# Autodesk Inventor assembly: Toolhead
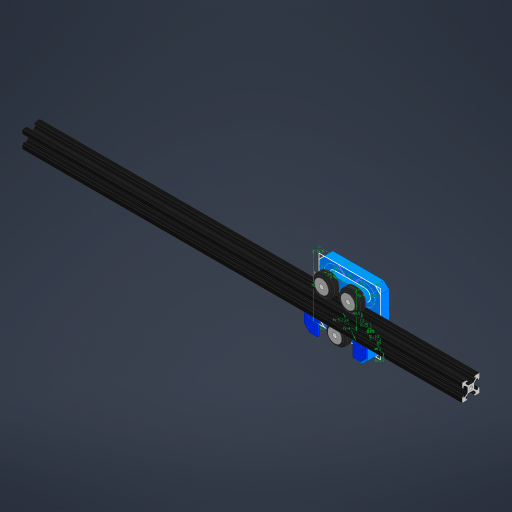
[picture p0: Inventor's stored thumbnail of the model, 512x512]
Saved by Autodesk Inventor 2024.2 (Build 282272000, 272)
## iProperties
Created: 2024-10-17
Part Number: Toolhead
Document SubType Name: Assembly
Designer: jerem
Author: jerem
## Documents named in this file (5)
- C:\Users\jerem\Documents\GitHub\Perovskite-Automated-Synthesis-System\CAD\Gantry\Toolhead\Toolhead.iam
- C:\Users\jerem\Documents\GitHub\Perovskite-Automated-Synthesis-System\CAD\Gantry\Extrusion\V Extrustion 20x500mm.ipt
- C:\Users\jerem\Documents\GitHub\Perovskite-Automated-Synthesis-System\CAD\Gantry\Printer Wheel.ipt
- C:\Users\jerem\Documents\GitHub\Perovskite-Automated-Synthesis-System\CAD\Gantry\Toolhead\Toolhead Base.ipt
- C:\Users\jerem\Documents\GitHub\Perovskite-Automated-Synthesis-System\CAD\Gantry\Toolhead\Belt Holders.ipt
## Components (7 placed, 4 different names)
1. V Extrustion 20x500mm:1 — Mate:7, Flush:1
2. Printer Wheel:1 — Mate:2, Mate:5
3. Printer Wheel:2 — Mate:3, Mate:6, Mate:7
4. Printer Wheel:3 — Mate:1, Mate:4
5. Toolhead Base:1 — Mate:1, Mate:2, Mate:3, Mate:4, Mate:5, Mate:6, Flush:1, Mate:8, Mate:9, Mate:10, Mate:11, Mate:12, Mate:13
6. Belt Holders:1 — Mate:8, Mate:9, Mate:10
7. Belt Holders:2 — Mate:11, Mate:12, Mate:13
## Relationships (14: Mate 13, Flush 1)
- Mate:1: Printer Wheel:3 ↔ Toolhead Base:1
- Mate:2: Printer Wheel:1 ↔ Toolhead Base:1
- Mate:3: Printer Wheel:2 ↔ Toolhead Base:1
- Mate:4: Printer Wheel:3 ↔ Toolhead Base:1
- Mate:5: Printer Wheel:1 ↔ Toolhead Base:1
- Mate:6: Printer Wheel:2 ↔ Toolhead Base:1
- Mate:7: V Extrustion 20x500mm:1 ↔ Printer Wheel:2
- Flush:1: V Extrustion 20x500mm:1 ↔ Toolhead Base:1
- Mate:8: Toolhead Base:1 ↔ Belt Holders:1
- Mate:9: Toolhead Base:1 ↔ Belt Holders:1
- Mate:10: Toolhead Base:1 ↔ Belt Holders:1
- Mate:11: Toolhead Base:1 ↔ Belt Holders:2
- Mate:12: Toolhead Base:1 ↔ Belt Holders:2
- Mate:13: Toolhead Base:1 ↔ Belt Holders:2
